# Autodesk Inventor assembly: EnsamblajeBarco
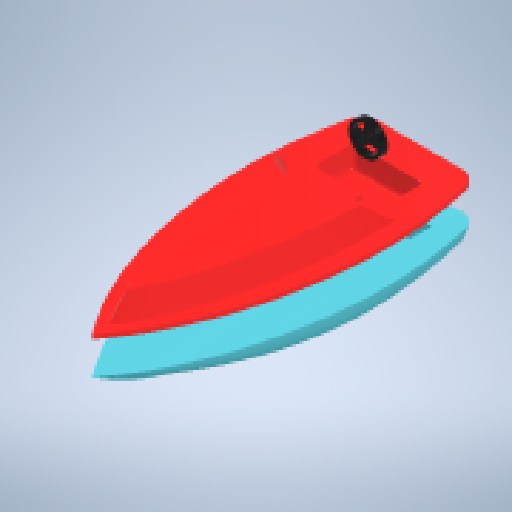
[picture p0: Inventor's stored thumbnail of the model, 512x512]
Saved by Autodesk Inventor 2025.1 (Build 291241000, 241)
## iProperties
Created: 2025-01-21
Part Number: EnsamblajeBarco
Document SubType Name: Assembly
Designer: usuario
Author: usuario
## Documents named in this file (5)
- C:\Users\yovan\Desktop\APM\ausol-apm.github.io\project\Design and simulation\Inventor\Modelado juguetes\Cad Juguetes\Barco\EnsamblajeBarco.iam
- C:\Users\yovan\Desktop\APM\ausol-apm.github.io\project\Design and simulation\Inventor\Modelado juguetes\Cad Juguetes\Barco\PiezabarcoInferior.ipt
- C:\Users\yovan\Desktop\APM\ausol-apm.github.io\project\Design and simulation\Inventor\Modelado juguetes\Cad Juguetes\Barco\Piezabarcosuperior.ipt
- C:\Users\yovan\Desktop\APM\ausol-apm.github.io\project\Design and simulation\Inventor\Modelado juguetes\Cad Juguetes\Barco\PiezaEjeTimon.ipt
- C:\Users\yovan\Desktop\APM\ausol-apm.github.io\project\Design and simulation\Inventor\Modelado juguetes\Cad Juguetes\Barco\PiezaTimon.ipt
## Components (4 placed, 4 different names)
1. PiezabarcoInferior:1 — Mate:1, Mate:2, Mate:3
2. Piezabarcosuperior:1 — Mate:1, Mate:2, Mate:3, Mate:4, Mate:5, Mate:6
3. PiezaEjeTimon:1 — Mate:4, Mate:5, Mate:6, Mate:7, Mate:8
4. PiezaTimon:1 — Mate:7, Mate:8
## Relationships (8: Mate 8)
- Mate:1 (15 mm): PiezabarcoInferior:1 ↔ Piezabarcosuperior:1
- Mate:2: PiezabarcoInferior:1 ↔ Piezabarcosuperior:1
- Mate:3: PiezabarcoInferior:1 ↔ Piezabarcosuperior:1
- Mate:4 (23 mm): Piezabarcosuperior:1 ↔ PiezaEjeTimon:1
- Mate:5: Piezabarcosuperior:1 ↔ PiezaEjeTimon:1
- Mate:6: Piezabarcosuperior:1 ↔ PiezaEjeTimon:1
- Mate:7: PiezaEjeTimon:1 ↔ PiezaTimon:1
- Mate:8: PiezaEjeTimon:1 ↔ PiezaTimon:1
